# Autodesk Inventor assembly: Wózek_inwalidzki
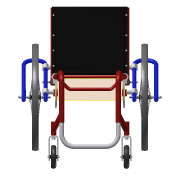
[picture p0: Inventor's stored thumbnail of the model, 180x180]
Saved by Autodesk Inventor 2015 (Build 190159000, 159)
## iProperties
Created: 2016-01-12
Part Number: Wózek_inwalidzki
Document SubType Name: Assembly
Designer: graaapsik
Author: graaapsik
## Documents named in this file (22)
- C:\Users\EriveltonDell\Documents\Centro Universitário da FEI\Wheelchair\CADEIRA DE RODAS - DESENHO\GITHUB\Wózek_inwalidzki.iam
- C:\Users\EriveltonDell\Documents\Centro Universitário da FEI\Wheelchair\CADEIRA DE RODAS - DESENHO\lasteverision\Power-Assisted-Wheelchair-master\Hamulec.iam
- C:\Users\EriveltonDell\Documents\Centro Universitário da FEI\Wheelchair\CADEIRA DE RODAS - DESENHO\lasteverision\Power-Assisted-Wheelchair-master\Koło_przednie.iam
- C:\Users\EriveltonDell\Documents\Centro Universitário da FEI\Wheelchair\CADEIRA DE RODAS - DESENHO\lasteverision\Power-Assisted-Wheelchair-master\Koło_tylne.iam
- C:\Users\EriveltonDell\Documents\Centro Universitário da FEI\Wheelchair\CADEIRA DE RODAS - DESENHO\lasteverision\Power-Assisted-Wheelchair-master\Rama_wozka.iam
- C:\Users\EriveltonDell\Documents\Centro Universitário da FEI\Wheelchair\CADEIRA DE RODAS - DESENHO\lasteverision\Power-Assisted-Wheelchair-master\Tapicerka_oparcia.iam
- C:\Users\EriveltonDell\Documents\Centro Universitário da FEI\Wheelchair\CADEIRA DE RODAS - DESENHO\lasteverision\Power-Assisted-Wheelchair-master\Tapicerka_siedziska.iam
- C:\Users\EriveltonDell\Documents\Centro Universitário da FEI\Wheelchair\CADEIRA DE RODAS - DESENHO\lasteverision\Power-Assisted-Wheelchair-master\Ciąg.iam
- C:\Users\EriveltonDell\Documents\Centro Universitário da FEI\Wheelchair\CADEIRA DE RODAS - DESENHO\lasteverision\Power-Assisted-Wheelchair-master\Widelec.iam
- C:\Users\EriveltonDell\Documents\Centro Universitário da FEI\Wheelchair\CADEIRA DE RODAS - DESENHO\lasteverision\Power-Assisted-Wheelchair-master\Zaślepka_do_widelca.ipt
- C:\Users\EriveltonDell\Documents\Centro Universitário da FEI\Wheelchair\CADEIRA DE RODAS - DESENHO\lasteverision\Power-Assisted-Wheelchair-master\Podnóżek.iam
- C:\Users\EriveltonDell\Documents\Centro Universitário da FEI\Wheelchair\CADEIRA DE RODAS - DESENHO\lasteverision\Power-Assisted-Wheelchair-master\Zaślepka_do_rur_fi32.ipt
- C:\Users\EriveltonDell\Documents\Centro Universitário da FEI\Wheelchair\CADEIRA DE RODAS - DESENHO\lasteverision\Power-Assisted-Wheelchair-master\GARFO.ipt
- C:\Users\EriveltonDell\Documents\Centro Universitário da FEI\Wheelchair\CADEIRA DE RODAS - DESENHO\lasteverision\Power-Assisted-Wheelchair-master\suporte-rodas-esq.ipt
- C:\Users\EriveltonDell\Documents\Centro Universitário da FEI\Wheelchair\CADEIRA DE RODAS - DESENHO\lasteverision\Power-Assisted-Wheelchair-master\suporte-rodas.ipt
- C:\Users\EriveltonDell\Documents\Centro Universitário da FEI\Wheelchair\CADEIRA DE RODAS - DESENHO\lasteverision\Power-Assisted-Wheelchair-master\suporte-eixo.ipt
- C:\Users\EriveltonDell\Documents\Centro Universitário da FEI\Wheelchair\CADEIRA DE RODAS - DESENHO\lasteverision\Power-Assisted-Wheelchair-master\suporte-barra.ipt
- C:\Users\EriveltonDell\Documents\Centro Universitário da FEI\Wheelchair\CADEIRA DE RODAS - DESENHO\lasteverision\Power-Assisted-Wheelchair-master\Barra-garfo.ipt
- C:\Users\EriveltonDell\Documents\Centro Universitário da FEI\Wheelchair\CADEIRA DE RODAS - DESENHO\lasteverision\Power-Assisted-Wheelchair-master\suporte-eixo - 2.ipt
- C:\Users\EriveltonDell\Documents\Centro Universitário da FEI\Wheelchair\CADEIRA DE RODAS - DESENHO\GITHUB\suporte-barra 2.ipt
- C:\Users\EriveltonDell\Documents\Centro Universitário da FEI\Wheelchair\CADEIRA DE RODAS - DESENHO\lasteverision\Power-Assisted-Wheelchair-master\ISO 4032 - M12ISO.ipt
- C:\Users\EriveltonDell\Documents\Centro Universitário da FEI\Wheelchair\CADEIRA DE RODAS - DESENHO\lasteverision\Power-Assisted-Wheelchair-master\ISO 4032 - M8ISO.ipt
## Components (40 placed, 22 different names)
1. Rama_wozka:1 [sub-assembly] — Zestawiający:7, Zestawiający:8, Zestawiający:9, Zestawiający:10, Zestawiający:11, Zestawiający:12, Równoległy:1, Zestawiający:15, Symetria:1, Równoległy:2, Zestawiający:20, Zestawiający:22, Zestawiający:27, Zestawiający:29, Zestawiający:36, Zestawiający:37, Równoległy:3, Zestawiający:38, Zestawiający:39, Zestawiający:40, Zestawiający:41, Zestawiający:42, Zestawiający:43, Zestawiający:44, Zestawiający:45, Angle:5, 49.15, Angle:9, Insert:13, Insert:14, Angle:12, Angle:13, Angle:14, Insert:30, Insert:31, Mate:63, Tangent:23, Angle:18, Tangent:24, Mate:64
2. Roda [sub-assembly] — Zestawiający:24, Zestawiający:25, Kąt:1, Angle:14, Mate:58, Mate:59, Mate:66
3. Koło_tylne:2 [sub-assembly] — Zestawiający:30, Zestawiający:31, Kąt:2, Angle:13, Mate:56, Mate:57, Angle:19, Mate:67
4. Ciąg:1 [sub-assembly] — Zestawiający:30, Zestawiający:31
5. Ciąg:2 [sub-assembly] — Zestawiający:24, Zestawiający:25
6. Widelec:1 [sub-assembly] — Zestawiający:9, Zestawiający:11, Wstaw:3
7. Widelec:2 [sub-assembly] — Zestawiający:10, Zestawiający:12, Zestawiający:13, Zestawiający:14, Symetria:1
8. Koło_przednie:1 [sub-assembly] — Wstaw:3, Kąt:1
9. Koło_przednie:2 [sub-assembly] — Zestawiający:13, Zestawiający:14, Kąt:2
10. Hamulec:1 [sub-assembly] — Zestawiający:38, Zestawiający:39, Angle:9
11. Tapicerka_oparcia:1 [sub-assembly] — Równoległy:1, Zestawiający:16
12. Tapicerka_siedziska:1 [sub-assembly] — Zestawiający:15, Zestawiający:16, Angle:10, Angle:11
13. Zaślepka_do_widelca:1 — Zestawiający:8, Zestawiający:45
14. Zaślepka_do_widelca:2 — Zestawiający:7, Zestawiający:44
15. Podnóżek:1 [sub-assembly] — Zestawiający:36, Zestawiający:37, Równoległy:3
16. Zaślepka_do_rur_fi32:1 — Zestawiający:22, Zestawiający:42
17. Zaślepka_do_rur_fi32:2 — Zestawiający:27, Zestawiający:40
18. Zaślepka_do_rur_fi32:3 — Zestawiający:20, Zestawiający:43
19. Zaślepka_do_rur_fi32:5 — Zestawiający:29, Zestawiający:41
20. GARFO:1 — Angle:5, Insert:24, Mate:58, Mate:59, Insert:28, Tangent:25, Tangent:27, Tangent:28
21. GARFO:2 — 49.15, Angle:15, Mate:56, Mate:57, Insert:25, Insert:29, Tangent:26, Tangent:29, Tangent:30
22. suporte-rodas-esq:1 — Insert:14, Angle:10, Mate:55, Tangent:19, Tangent:20
23. suporte-rodas:1 — Insert:13, Angle:11, Mate:62, Tangent:21, Tangent:22
24. suporte-eixo:2 — Mate:55, Tangent:19, Tangent:20, Mate:60, Mate:61
25. suporte-barra:1 — Insert:22, Insert:24, Angle:17
26. suporte-barra:2 — Angle:15, Angle:16, Insert:29
27. Barra-garfo:1 — Angle:12, Insert:22
28. suporte-barra:3 — Insert:28, Angle:17, Mate:65
29. suporte-barra:4 — Insert:25, Angle:16, Mate:60, Mate:61
30. suporte-eixo - 2:1 — Mate:62, Tangent:21, Tangent:22, Mate:65
31. Zaślepka_do_rur_fi32:6 — Insert:30
32. Zaślepka_do_rur_fi32:7 — Insert:31
33. suporte-barra 2:1 — Mate:63, Tangent:23, Angle:18, Mate:68, Mate:69
34. suporte-barra 2:2 — Tangent:24, Mate:64, Angle:19, Mate:70, Mate:71
35. ISO 4032 M12:1 — Mate:66, Tangent:25
36. ISO 4032 M12:2 — Mate:67, Tangent:26
37. ISO 4032 M8:1 — Mate:71, Tangent:30
38. ISO 4032 M8:2 — Mate:70, Tangent:29
39. ISO 4032 M8:3 — Mate:69, Tangent:28
40. ISO 4032 M8:4 — Mate:68, Tangent:27
## Relationships (86: Mate 45, Angle 15, Tangent 12, Insert 10, Flush 3, Symmetry 1)
- Zestawiający:7 [Mate]: Rama_wozka:1 ↔ Zaślepka_do_widelca:2
- Zestawiający:8 [Mate]: Rama_wozka:1 ↔ Zaślepka_do_widelca:1
- Zestawiający:9 [Mate]: Rama_wozka:1 ↔ Widelec:1
- Zestawiający:10 [Mate]: Rama_wozka:1 ↔ Widelec:2
- Zestawiający:11 [Mate]: Rama_wozka:1 ↔ Widelec:1
- Zestawiający:12 [Mate]: Rama_wozka:1 ↔ Widelec:2
- Zestawiający:13 [Mate]: Widelec:2 ↔ Koło_przednie:2
- Zestawiający:14 [Mate]: Widelec:2 ↔ Koło_przednie:2
- Równoległy:1 [Flush] (-16 mm): Rama_wozka:1 ↔ Tapicerka_oparcia:1
- Zestawiający:15 [Mate] (16 mm): Rama_wozka:1 ↔ Tapicerka_siedziska:1
- Zestawiający:16 [Mate] (0.25 mm): Tapicerka_oparcia:1 ↔ Tapicerka_siedziska:1
- Symetria:1 [Symmetry]: Rama_wozka:1 ↔ Widelec:2
- Równoległy:2 [Flush]: Rama_wozka:1
- Zestawiający:20 [Mate]: Rama_wozka:1 ↔ Zaślepka_do_rur_fi32:3
- Zestawiający:22 [Mate]: Rama_wozka:1 ↔ Zaślepka_do_rur_fi32:1
- Zestawiający:24 [Mate]: Roda ↔ Ciąg:2
- Zestawiający:25 [Mate]: Roda ↔ Ciąg:2
- Zestawiający:27 [Mate]: Rama_wozka:1 ↔ Zaślepka_do_rur_fi32:2
- Zestawiający:29 [Mate]: Rama_wozka:1 ↔ Zaślepka_do_rur_fi32:5
- Zestawiający:30 [Mate]: Koło_tylne:2 ↔ Ciąg:1
- Zestawiający:31 [Mate]: Koło_tylne:2 ↔ Ciąg:1
- Wstaw:3 [Insert]: Widelec:1 ↔ Koło_przednie:1
- Zestawiający:36 [Mate]: Rama_wozka:1 ↔ Podnóżek:1
- Zestawiający:37 [Mate]: Rama_wozka:1 ↔ Podnóżek:1
- Równoległy:3 [Flush] (150 mm): Rama_wozka:1 ↔ Podnóżek:1
- Zestawiający:38 [Mate]: Rama_wozka:1 ↔ Hamulec:1
- Zestawiający:39 [Mate] (40 mm): Rama_wozka:1 ↔ Hamulec:1
- Zestawiający:40 [Mate]: Rama_wozka:1 ↔ Zaślepka_do_rur_fi32:2
- Zestawiający:41 [Mate]: Rama_wozka:1 ↔ Zaślepka_do_rur_fi32:5
- Zestawiający:42 [Mate]: Rama_wozka:1 ↔ Zaślepka_do_rur_fi32:1
- Zestawiający:43 [Mate]: Rama_wozka:1 ↔ Zaślepka_do_rur_fi32:3
- Zestawiający:44 [Mate]: Rama_wozka:1 ↔ Zaślepka_do_widelca:2
- Zestawiający:45 [Mate]: Rama_wozka:1 ↔ Zaślepka_do_widelca:1
- Kąt:1 [Angle] (0 deg): Roda ↔ Koło_przednie:1
- Kąt:2 [Angle] (0 deg): Koło_tylne:2 ↔ Koło_przednie:2
- Angle:5 (126 deg): Rama_wozka:1 ↔ GARFO:1
- 49.15 [Angle] (54 deg): Rama_wozka:1 ↔ GARFO:2
- Angle:9 (0 deg): Rama_wozka:1 ↔ Hamulec:1
- Insert:13 (150 mm): Rama_wozka:1 ↔ suporte-rodas:1
- Insert:14 (150 mm): Rama_wozka:1 ↔ suporte-rodas-esq:1
- Angle:10 (90 deg): Tapicerka_siedziska:1 ↔ suporte-rodas-esq:1
- Angle:11 (90 deg): Tapicerka_siedziska:1 ↔ suporte-rodas:1
- Mate:55: suporte-rodas-esq:1 ↔ suporte-eixo:2
- Tangent:19: suporte-rodas-esq:1 ↔ suporte-eixo:2
- Tangent:20: suporte-rodas-esq:1 ↔ suporte-eixo:2
- Angle:12 (0 deg): Rama_wozka:1 ↔ Barra-garfo:1
- Angle:13 (0 deg): Rama_wozka:1 ↔ Koło_tylne:2
- Angle:14 (0 deg): Rama_wozka:1 ↔ Roda
- Insert:22: suporte-barra:1 ↔ Barra-garfo:1
- Angle:15 (0 deg): GARFO:2 ↔ suporte-barra:2
- Mate:56 (10 mm): Koło_tylne:2 ↔ GARFO:2
- Mate:57: Koło_tylne:2 ↔ GARFO:2
- Insert:24: GARFO:1 ↔ suporte-barra:1
- Mate:58: Roda ↔ GARFO:1
- Mate:59 (10 mm): Roda ↔ GARFO:1
- Insert:25 (-100 mm): GARFO:2 ↔ suporte-barra:4
- Angle:16 (0 deg): suporte-barra:2 ↔ suporte-barra:4
- Mate:60: suporte-eixo:2 ↔ suporte-barra:4
- Mate:61: suporte-eixo:2 ↔ suporte-barra:4
- Mate:62: suporte-rodas:1 ↔ suporte-eixo - 2:1
- Insert:28 (-100 mm): GARFO:1 ↔ suporte-barra:3
- Angle:17 (0 deg): suporte-barra:1 ↔ suporte-barra:3
- Insert:29: GARFO:2 ↔ suporte-barra:2
- Tangent:21: suporte-rodas:1 ↔ suporte-eixo - 2:1
- Tangent:22: suporte-rodas:1 ↔ suporte-eixo - 2:1
- Insert:30 (-8 mm): Rama_wozka:1 ↔ Zaślepka_do_rur_fi32:6
- Insert:31 (-8 mm): Rama_wozka:1 ↔ Zaślepka_do_rur_fi32:7
- Mate:63: Rama_wozka:1 ↔ suporte-barra 2:1
- Tangent:23: Rama_wozka:1 ↔ suporte-barra 2:1
- Angle:18 (0 deg): Rama_wozka:1 ↔ suporte-barra 2:1
- Tangent:24: Rama_wozka:1 ↔ suporte-barra 2:2
- Mate:64: Rama_wozka:1 ↔ suporte-barra 2:2
- Angle:19 (0 deg): Koło_tylne:2 ↔ suporte-barra 2:2
- Mate:65: suporte-barra:3 ↔ suporte-eixo - 2:1
- Mate:66: Roda ↔ ISO 4032 M12:1
- Tangent:25: GARFO:1 ↔ ISO 4032 M12:1
- Mate:67: Koło_tylne:2 ↔ ISO 4032 M12:2
- Tangent:26: GARFO:2 ↔ ISO 4032 M12:2
- Mate:68: suporte-barra 2:1 ↔ ISO 4032 M8:4
- Tangent:27: GARFO:1 ↔ ISO 4032 M8:4
- Mate:69: suporte-barra 2:1 ↔ ISO 4032 M8:3
- Tangent:28: GARFO:1 ↔ ISO 4032 M8:3
- Mate:70: suporte-barra 2:2 ↔ ISO 4032 M8:2
- Tangent:29: GARFO:2 ↔ ISO 4032 M8:2
- Mate:71: suporte-barra 2:2 ↔ ISO 4032 M8:1
- Tangent:30: GARFO:2 ↔ ISO 4032 M8:1
## Named parameters: sa_0 = 1.6e-12, sa_1 = -6.84e-11, sa_2 = -70000
note: some values were not read from the file. Shown as the stored number, unit unknown: "sa_0", "sa_1", "sa_2".
